# Autodesk Inventor assembly: UmlenkrolleHalterHeavy
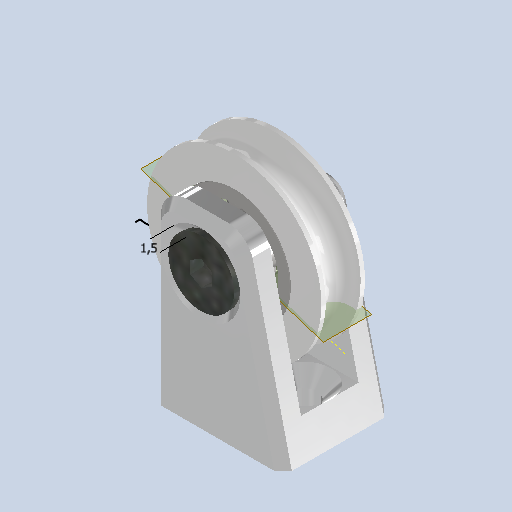
[picture p0: Inventor's stored thumbnail of the model, 512x512]
Saved by Autodesk Inventor 2025 (Build 290162010, 162A)
## iProperties
Created: 2024-11-19
Part Number: UmlenkrolleHalterHeavy
Document SubType Name: Assembly
Designer: Admin
Author: Admin
## Documents named in this file (5)
- C:\Users\Admin\GIT\HDVKBM\CAD\Krandemonstrator\UmlenkrolleHalterHeavy.iam
- C:\Users\Admin\GIT\HDVKBM\CAD\Krandemonstrator\Umlenkrolle.iam
- C:\Users\Admin\GIT\HDVKBM\CAD\Krandemonstrator\HalterUmlenkrolleH.ipt
- C:\Users\Admin\Documents\Inventor\Content Center Files\R2025\de-DE\DIN EN ISO 7089\DIN EN ISO 7089 -  4.ipt
- C:\Users\Admin\Documents\Inventor\Content Center Files\R2025\de-DE\ISO 10642(2)\ISO 10642  - M4  x  12.ipt
## Components (5 placed, 4 different names)
1. HalterUmlenkrolleH:1
2. Umlenkrolle:1 [sub-assembly] — Drehbar:1
3. DIN EN ISO 7089 4:1
4. DIN EN ISO 7089 4:2 — Drehbar:1
5. DIN EN ISO 10642 M4  x  12:1
## Relationships (4: WeldJoint 2, Mate 1, RevoluteJoint 1)
- [WeldJoint]: HalterUmlenkrolleH:1 ↔ DIN EN ISO 7089 4:1
- [Mate]: HalterUmlenkrolleH:1 ↔ DIN EN ISO 10642 M4  x  12:1
- [WeldJoint]: HalterUmlenkrolleH:1 ↔ DIN EN ISO 7089 4:2
- Drehbar:1 [RevoluteJoint]: Umlenkrolle:1 ↔ DIN EN ISO 7089 4:2
